# Autodesk Inventor assembly: Arm 2.0 Assembly
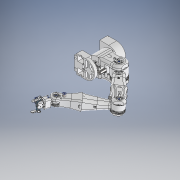
[picture p0: Inventor's stored thumbnail of the model, 180x180]
Saved by Autodesk Inventor 2017 SP1 (Build 210196100, 196)
## iProperties
Created: 2017-09-28
Part Number: Arm 2.0 Assembly
Document SubType Name: Assembly
Designer: Zach
Author: Zach
## Documents named in this file (62)
- C:\Users\Zach\Documents\GitHub\tr1\src\Body\Arm 2.0 Assembly\Arm 2.0 Assembly.iam
- C:\Users\Zach\Documents\GitHub\tr1\src\Body\Arm 2.0 Assembly\Steel Rod 8mm x 135mm.ipt
- C:\Users\Zach\Documents\GitHub\tr1\lib\22x8x8mm Bearing.ipt
- C:\Users\Zach\Documents\GitHub\tr1\src\Body\Arm 2.0 Assembly\AA004.ipt
- C:\Users\Zach\Documents\GitHub\tr1\lib\QS12MM250\QS12MM250.ipt
- C:\Users\Zach\Documents\GitHub\tr1\src\Body\Arm 2.0 Assembly\Steel Rod 8mm x 100mm.ipt
- C:\Users\Zach\Documents\GitHub\tr1\src\Body\Arm 2.0 Assembly\AA013.ipt
- C:\Users\Zach\Documents\GitHub\tr1\src\Body\Arm 2.0 Assembly\AA014.ipt
- C:\Users\Zach\Documents\GitHub\tr1\lib\12V DC Motor 378-1.ipt
- C:\Users\Zach\Documents\Inventor\Content Center Files\R2017\en-US\ISO 4017(1)\ISO 4017 - M5 x 20 - ISO.ipt
- C:\Users\Zach\Documents\GitHub\tr1\src\Body\Arm 2.0 Assembly\Steel Rod 8mm x 80mm.ipt
- C:\Users\Zach\Documents\GitHub\BCN3D-Moveo\Autodesk Inventor files\Gripper B Assembly.iam
- C:\Users\Zach\Documents\Inventor\Content Center Files\R2017\en-US\CNS 4320\CNS 4320 - M8 x 1 x 100.ipt
- C:\Users\Zach\Documents\GitHub\tr1\lib\AS 1110 - M8 x 150.ipt
- C:\Users\Zach\Documents\GitHub\tr1\lib\8mm Hub.ipt
- C:\Users\Zach\Documents\GitHub\tr1\src\Body\Arm 2.0 Assembly\Arm 2.0 Assembly\Design Accelerator\Spur Gears5.iam
- C:\Users\Zach\Documents\GitHub\tr1\lib\4mm mounting hub.ipt
- C:\Users\Zach\Documents\GitHub\tr1\lib\6201RS\6201RS.ipt
- C:\Users\Zach\Documents\GitHub\tr1\lib\U51105\U51105.ipt
- C:\Users\Zach\Documents\GitHub\tr1\src\Body\Arm 2.0 Assembly\AA031.ipt
- C:\Users\Zach\Documents\GitHub\tr1\src\Body\Arm 2.0 Assembly\AA034.ipt
- C:\Users\Zach\Documents\GitHub\tr1\src\Body\Arm 2.0 Assembly\Arm 2.0 Assembly\Design Accelerator\Spur Gears6.iam
- C:\Users\Zach\Documents\GitHub\tr1\src\Body\Arm 2.0 Assembly\AA008c.ipt
- C:\Users\Zach\Documents\GitHub\tr1\src\Body\Arm 2.0 Assembly\AA008d.ipt
- C:\Users\Zach\Documents\GitHub\tr1\src\Body\Arm 2.0 Assembly\AA035.ipt
- C:\Users\Zach\Documents\GitHub\tr1\src\Body\Arm 2.0 Assembly\Arm 2.0 Assembly\Design Accelerator\Spur Gears7.iam
- C:\Users\Zach\Documents\GitHub\tr1\src\Body\Arm 2.0 Assembly\AA036.ipt
- C:\Users\Zach\Documents\GitHub\tr1\src\Body\Arm 2.0 Assembly\AA037.ipt
- C:\Users\Zach\Documents\GitHub\tr1\src\Body\Arm 2.0 Assembly\AA016b.ipt
- C:\Users\Zach\Documents\GitHub\tr1\src\Body\Arm 2.0 Assembly\AA005b.ipt
- C:\Users\Zach\Documents\GitHub\tr1\src\Body\Arm 2.0 Assembly\AA006b.ipt
- C:\Users\Zach\Documents\GitHub\tr1\src\Body\Arm 2.0 Assembly\AA001c.ipt
- C:\Users\Zach\Documents\GitHub\tr1\lib\uxcell 12V 5RPM 8mm Worm Gear Motor\uxcell 12V 5RPM 8mm Worm Gear Motor.ipt
- C:\Users\Zach\Documents\GitHub\tr1\lib\Bourns ACE 128\Bourns ACE 128.ipt
- C:\Users\Zach\Documents\GitHub\tr1\src\Body\Arm 2.0 Assembly\Arm 2.0 Assembly\Design Accelerator\Spur Gears8.iam
- C:\Users\Zach\Documents\GitHub\tr1\src\Body\Arm 2.0 Assembly\Arm 2.0 Assembly\Design Accelerator\Spur Gears11.iam
- C:\Users\Zach\Documents\GitHub\tr1\src\Body\Arm 2.0 Assembly\Arm 2.0 Assembly\Design Accelerator\Spur Gears9.iam
- C:\Users\Zach\Documents\GitHub\tr1\src\Body\Arm 2.0 Assembly\AA010b.ipt
- C:\Users\Zach\Documents\GitHub\tr1\lib\uxcell 12V 6RPM 6mm Worm Gear Motor\uxcell 12V 6RPM 6mm Worm Gear Motor.ipt
- C:\Users\Zach\Documents\GitHub\tr1\src\Body\Arm 2.0 Assembly\Arm 2.0 Assembly\Design Accelerator\Spur Gears10.iam
- C:\Users\Zach\Documents\GitHub\tr1\src\Body\Arm 2.0 Assembly\Arm 2.0 Assembly\Design Accelerator\Spur Gears12.iam
- C:\Users\Zach\Documents\GitHub\tr1\src\Body\Arm 2.0 Assembly\AA041.ipt
- C:\Users\Zach\Documents\GitHub\tr1\src\Body\Arm 2.0 Assembly\AA042.ipt
- C:\Users\Zach\Documents\Inventor\Content Center Files\R2017\en-US\ISO 7045  H\ISO 7045 - M3 x 8 - 4.8 - H - ISO.ipt
- C:\Users\Zach\Documents\GitHub\tr1\src\Body\Arm 2.0 Assembly\AA043.ipt
- C:\Users\Zach\Documents\GitHub\tr1\src\Body\Arm 2.0 Assembly\AA044.ipt
- C:\Users\Zach\Documents\GitHub\tr1\src\Body\Arm 2.0 Assembly\AA045.ipt
- C:\Users\Zach\Documents\GitHub\tr1\src\Body\Arm 2.0 Assembly\Arm 2.0 Assembly\Design Accelerator\Spur Gears13.iam
- C:\Users\Zach\Documents\GitHub\tr1\src\Body\Arm 2.0 Assembly\Arm 2.0 Assembly\Design Accelerator\Spur Gears16.iam
- C:\Users\Zach\Documents\GitHub\tr1\src\Body\Arm 2.0 Assembly\AA046.ipt
- C:\Users\Zach\Documents\GitHub\tr1\lib\MG995.ipt
- C:\Users\Zach\Documents\GitHub\tr1\lib\Servo Mounting Hub.ipt
- C:\Users\Zach\Documents\GitHub\tr1\src\Body\Arm 2.0 Assembly\AA047.ipt
- C:\Users\Zach\Documents\GitHub\tr1\src\Body\Arm 2.0 Assembly\AA048.ipt
- C:\Users\Zach\Documents\Inventor\Content Center Files\R2017\en-US\ISO 4018\ISO 4018 - M5 x 10.ipt
- C:\Users\Zach\Documents\Inventor\Content Center Files\R2017\en-US\ISO 4018\ISO 4018 - M5 x 25.ipt
- C:\Users\Zach\Documents\Inventor\Content Center Files\R2017\en-US\ISO 7045  H\ISO 7045 - M3 x 12 - 4.8 - H - ISO.ipt
- C:\Users\Zach\Documents\GitHub\tr1\src\Body\Arm 2.0 Assembly\AA049.ipt
- C:\Users\Zach\Documents\Inventor\Content Center Files\R2017\en-US\ISO 4018\ISO 4018 - M5 x 40.ipt
- C:\Users\Zach\Documents\Inventor\Content Center Files\R2017\en-US\ISO 4035(2)\ISO 4035 - M5 - ISO.ipt
- C:\Users\Zach\Documents\Inventor\Content Center Files\R2017\en-US\ISO 4018\ISO 4018 - M5 x 35.ipt
- C:\Users\Zach\Documents\Inventor\Content Center Files\R2017\en-US\ISO 4762(2)\ISO 4762 - M4 x 10ISO.ipt
## Components (204 placed, 61 different names)
1. AA001c:1 — Mate:554, Mate:555, Mate:556, Mate:557, Mate:560, Flush:18, Mate:562, Mate:563, Mate:564, Mate:565, Mate:566, Mate:567, Mate:568, Mate:569, Mate:570, Mate:571, Mate:572, Mate:573, Mate:574, Mate:576, Mate:578, Mate:581, Angle:1, Mate:592, Mate:602, Mate:834, Mate:835, Mate:836, Mate:837, Mate:895, Mate:905, Mate:906
2. AA004:1 — Mate:23, Mate:345, Mate:347, Mate:350, Mate:357, Mate:554, Mate:555, Mate:556, Mate:590, Mate:591, Mate:826
3. AA005b:1 — Mate:537, Mate:538, Mate:539, Mate:541, Mate:542, Mate:543, Mate:806, Mate:807, Mate:808, Mate:809, Mate:838, Mate:909, Mate:910
4. AA006b:1 — Mate:544, Mate:583, Mate:584, Angle:2, Mate:588, Mate:593, Mate:594, Mate:598, Mate:599, Mate:600, Mate:609, Mate:802, Mate:803, Mate:804, Mate:805, Mate:838
5. AA008c:1 — Mate:449, Mate:450, Mate:451, Mate:452, Mate:453, Mate:454, Mate:463, Mate:464, Mate:466, Mate:467, Mate:481, Mate:616, Mate:662, Mate:663, Mate:751
6. AA008d:1 — Mate:455, Mate:456, Mate:457, Mate:461, Mate:463, Mate:464, Mate:466, Mate:467, Mate:614, Angle:4, Mate:635, Mate:662, Mate:663, Mate:697, Mate:699, Mate:751, Mate:846, Mate:847, Mate:848, Mate:849, Mate:854, Mate:855, Mate:856, Mate:857, Flush:22, Flush:23, Mate:858, Mate:859, Mate:925, Mate:926
7. AA010b:1 — Mate:615, Mate:616, Mate:617, Mate:618, Mate:620, Mate:621, Mate:623, Mate:624, Mate:625, Mate:626, Mate:628, Mate:630, Mate:632, Mate:633, Mate:634, Mate:636, Mate:637, Angle:6, Mate:642, Flush:20, Mate:648, Mate:650, Mate:927, Mate:928, Mate:929, Mate:930, Mate:931, Mate:932, Mate:948, Mate:949
8. AA013:2 — Mate:142, Mate:143, Mate:144, Mate:145, Mate:146, Mate:147, Mate:563, Mate:564, Mate:565
9. AA014:2 — Mate:628, Mate:629, Mate:630, Mate:976, Mate:977, Mate:978, Mate:979, Mate:980, Mate:981
10. AA016b:1 — Mate:518, Mate:519, Mate:520, Mate:521, Mate:525, Mate:526, Mate:527, Mate:529, Mate:530, Mate:664, Mate:665, Mate:667, Mate:668, Mate:669, Angle:7, Mate:671, Mate:673, Mate:675, Mate:676, Mate:677, Mate:877, Mate:878
11. AA031:1 — Mate:366, Mate:367, Mate:523, Mate:524, Mate:954, Mate:955, Mate:956, Mate:957
12. AA034:1 — Mate:529, Mate:534, Mate:535, Mate:700, Mate:701, Mate:709, Mate:879, Mate:880, Mate:881, Mate:882, Mate:883, Mate:884, Mate:885, Mate:886, Mate:964, Mate:965, Mate:966, Mate:967, Mate:968, Mate:969, Mate:970, Mate:971, Mate:972, Mate:973, Mate:974, Mate:975
13. AA035:1 — Mate:477, Mate:479, Mate:481, Mate:557, Mate:601, Mate:652, Mate:653, Mate:697, Mate:699, Mate:851, Mate:853
14. AA036:1 — Mate:498, Mate:501, Mate:502, Mate:511, Mate:698, Mate:868, Mate:871, Mate:872, Mate:939
15. AA037:1 — Mate:501, Mate:502, Mate:514, Mate:515, Mate:516, Mate:517, Mate:518, Mate:519, Mate:520, Mate:530, Mate:664, Mate:665, Mate:698, Mate:866, Mate:867, Mate:873, Mate:874, Mate:875, Mate:876, Flush:25, Flush:26, Mate:950, Mate:951, Mate:952, Mate:953
16. AA041:1 — Mate:675, Mate:676, Mate:677, Mate:682, Mate:683, Mate:684, Mate:685
17. AA042:1 — Mate:678, Mate:679, Mate:686, Mate:687, Angle:14
18. AA043:1 — Mate:688, Mate:689, Angle:8
19. AA043:2 — Mate:693, Mate:694, Angle:10
20. AA043:3 — Mate:742, Mate:743, Angle:13
21. AA044:1 — Mate:691, Mate:692, Angle:9
22. AA044:2 — Mate:695, Mate:696, Angle:11, Mate:892, Mate:893
23. AA045:2 — Mate:700, Mate:701, Mate:702, Mate:703, Mate:704, Mate:705, Mate:706, Mate:708, Flush:21, Mate:709, Mate:711, Mate:713, Mate:715, Mate:717, Mate:718, Angle:12, Mate:719, Mate:720, Mate:723, Mate:725, Mate:780, Mate:781, Mate:784, Mate:785
24. AA046:1 — Mate:727, Mate:728, Mate:731, Mate:735, Mate:736, Mate:737, Mate:752, Mate:756, Mate:757, Mate:758, Mate:759, Mate:760, Mate:761, Mate:762, Mate:763
25. AA047:1 — Mate:735, Mate:736, Mate:737, Mate:738, Mate:739, Mate:740, Mate:753, Mate:754, Mate:755, Mate:800, Mate:801
26. AA048:1 — Mate:744, Mate:745, Mate:746, Mate:747, Mate:748, Mate:749
27. AA049:1 — Mate:783, Mate:784, Mate:785, Mate:786, Mate:787, Mate:788, Mate:789, Mate:790, Mate:791
28. Gripper B Assembly:1 [sub-assembly] — Mate:747, Mate:748, Mate:749
29. 22x8x8mm Bearing:1 — Mate:433, Mate:560
30. 22x8x8mm Bearing:2 — Mate:437, Mate:562
31. 22x8x8mm Bearing:3 — Mate:57, Mate:620, Mate:626, Mate:645
32. 22x8x8mm Bearing:4 — Mate:621, Mate:629, Mate:642
33. 22x8x8mm Bearing:5 — Mate:186, Mate:708
34. 22x8x8mm Bearing:6 — Mate:187, Mate:719
35. 22x8x8mm Bearing:7 — Mate:264, Mate:526
36. 22x8x8mm Bearing:8 — Mate:527, Mate:528
37. 22x8x8mm Bearing:13 — Mate:451, Mate:452
38. 22x8x8mm Bearing:14 — Mate:449, Mate:450
39. QS12MM250:1 — Mate:23, Mate:344, Mate:346, Mate:348, Mate:354, Mate:537, Mate:544, Mate:585, Mate:593, Mate:594, Mate:597
40. Steel Rod 8mm x 135mm:1 — Mate:433, Mate:437, Mate:476, Mate:477, Flush:18, Mate:575, Mate:651
41. Steel Rod 8mm x 100mm:1 — Mate:57, Mate:491, Mate:498, Flush:20, Mate:644, Mate:649
42. Steel Rod 8mm x 80mm:1 — Mate:186, Mate:187, Mate:706, Flush:21, Mate:710, Mate:721, Mate:724, Mate:730, Mate:783
43. 12V DC Motor 378-1:3 — Mate:702, Mate:703, Mate:704, Mate:705, Mate:712, Mate:714, Mate:778, Mate:779
44. 12V DC Motor 378-1:4 — Mate:514, Mate:515, Mate:516, Mate:522
45. 12V DC Motor 378-1:6 — Mate:340, Mate:342, Mate:538, Mate:539, Mate:540, Mate:543, Mate:907, Mate:908
46. 12V DC Motor 378-1:7 — Mate:455, Mate:456, Mate:457, Mate:460, Mate:610, Mate:923, Mate:924
47. uxcell 12V 6RPM 6mm Worm Gear Motor:1 — Mate:632, Mate:633, Mate:634, Mate:946, Mate:947
48. uxcell 12V 5RPM 8mm Worm Gear Motor:1 — Mate:568, Mate:569, Mate:570, Mate:571, Mate:572, Mate:894, Mate:903, Mate:904
49. 6201RS:1 — Mate:346, Mate:347
50. 6201RS:2 — Mate:357, Mate:597
51. U51105:1 — Mate:348, Mate:349, Mate:542
52. U51105:2 — Mate:354, Mate:608, Mate:609
53. 8mm Hub:2 — Mate:368, Mate:531, Mate:534, Mate:535
54. 8mm Hub:3 — Mate:617, Mate:618, Mate:690, Mate:933, Mate:934, Mate:935, Mate:936, Mate:937, Mate:938
55. 8mm Hub:4 — Mate:580, Mate:581, Mate:582
56. 8mm Hub:5 — Mate:644, Mate:645, Mate:646
57. 8mm Hub:6 — Mate:651, Mate:652, Mate:653, Mate:911, Mate:912, Mate:913, Mate:914, Mate:915, Mate:916
58. 8mm Hub:7 — Mate:666, Mate:667, Mate:674
59. 8mm Hub:8 — Mate:720, Mate:721, Mate:726
60. 8mm Hub:9 — Mate:727, Mate:728, Mate:730, Mate:756, Mate:764, Mate:765, Mate:766, Mate:767, Mate:768, Mate:769
61. 8mm Hub:10 — Mate:894, Mate:895, Mate:896
62. 4mm mounting hub:1 — Mate:340, Mate:540, Mate:541, Mate:887
63. 4mm mounting hub:3 — Mate:366, Mate:367, Mate:517, Mate:522, Mate:523, Mate:524
64. 4mm mounting hub:5 — Mate:513, Mate:622, Mate:623
65. 4mm mounting hub:7 — Mate:460, Mate:461, Mate:611, Mate:613
66. 4mm mounting hub:8 — Mate:714, Mate:715, Mate:716, Mate:782
67. Servo Mounting Hub:1 — Mate:733, Mate:734, Mate:738, Mate:739, Mate:740, Mate:792, Mate:793, Mate:794, Mate:795, Mate:796, Mate:797, Mate:798, Mate:799
68. Bourns ACE 128:1 — Mate:573, Mate:574, Mate:577, Angle:1, Mate:693, Mate:694
69. Bourns ACE 128:2 — Mate:583, Mate:584, Angle:2, Mate:587, Mate:695, Mate:696
70. Bourns ACE 128:3 — Mate:612, Mate:614, Angle:4, Mate:635, Mate:691, Mate:692
71. Bourns ACE 128:4 — Mate:636, Mate:637, Angle:6, Mate:647, Mate:688, Mate:689
72. Bourns ACE 128:5 — Mate:668, Mate:669, Angle:7, Mate:672, Mate:678, Mate:679
73. Bourns ACE 128:6 — Mate:717, Mate:718, Angle:12, Mate:722, Mate:742, Mate:743
74. AASG01 [sub-assembly] — Mate:342, Mate:344, Mate:345, Mate:349, Mate:350, Mate:810, Mate:811, Mate:812, Mate:813, Mate:814, Mate:815, Mate:816, Mate:817, Mate:818, Mate:819, Mate:820, Mate:821, Mate:887, Mate:888, Mate:889, Mate:890, Mate:891
75. AASG02 [sub-assembly] — Mate:476, Mate:479, Mate:566, Mate:567, Mate:601, Mate:602, Mate:839, Mate:841, Mate:842, Mate:843, Mate:844, Mate:845, Mate:896, Mate:897, Mate:898, Mate:899, Mate:900, Mate:901, Mate:902
76. AASG03 [sub-assembly] — Mate:491, Mate:511, Mate:513, Mate:622, Mate:624, Mate:625, Mate:860, Mate:861, Mate:862, Mate:863, Mate:864, Mate:865, Mate:940, Mate:941, Mate:942, Mate:943, Mate:944, Mate:945
77. AASG04 [sub-assembly] — Mate:575, Mate:576, Mate:577, Mate:578, Mate:580, Mate:582, Angle:10, Mate:917, Mate:918, Mate:919, Mate:920, Mate:921, Mate:922
78. AASG05 [sub-assembly] — Mate:585, Mate:587, Mate:588, Mate:590, Mate:591, Mate:592, Mate:608, Angle:11, Mate:822, Mate:823, Mate:824, Mate:825, Mate:827, Mate:828, Mate:829, Mate:830, Mate:831, Mate:832, Mate:833
79. AASG06 [sub-assembly] — Mate:610, Mate:611, Mate:612, Mate:613, Angle:5, Angle:9
80. AASG07 [sub-assembly] — Mate:646, Mate:647, Mate:648, Mate:649, Mate:650, Angle:8, Mate:958, Mate:959, Mate:960, Mate:961, Mate:962, Mate:963
81. AASG08 [sub-assembly] — Mate:670, Mate:671, Mate:672, Mate:673, Mate:674, Mate:680, Mate:681, Angle:14
82. AASG09 [sub-assembly] — Mate:710, Mate:711, Mate:712, Mate:713, Mate:716, Mate:731, Mate:757, Mate:770, Mate:771, Mate:772, Mate:773, Mate:774, Mate:775, Mate:776, Mate:777, Mate:782
83. AASG10 [sub-assembly] — Mate:722, Mate:723, Mate:724, Mate:725, Mate:726, Angle:13
84. MG995:1 — Mate:733, Mate:734, Mate:744, Mate:745, Mate:746
85. CNS 4320 M8 x 100:1 — Mate:264, Mate:368, Mate:521, Mate:525, Mate:528, Mate:531, Mate:666, Mate:670
86. AS 1110 - Metric M8 x 150:2 — Mate:453, Mate:454, Angle:5, Mate:615, Mate:690
87. ISO 7045 H M3 x 8 - 4.8 - H:1 — Mate:680, Mate:681
88. ISO 7045 H M3 x 8 - 4.8 - H:2 — Mate:682, Mate:685
89. ISO 7045 H M3 x 8 - 4.8 - H:3 — Mate:683, Mate:684
90. ISO 7045 H M3 x 8 - 4.8 - H:4 — Mate:686, Mate:687
91. ISO 7045 H M3 x 8 - 4.8 - H:5 — Mate:778, Mate:780
92. ISO 7045 H M3 x 8 - 4.8 - H:6 — Mate:779, Mate:781
93. ISO 7045 H M3 x 8 - 4.8 - H:7 — Mate:795, Mate:799
94. ISO 7045 H M3 x 8 - 4.8 - H:8 — Mate:794, Mate:798
95. ISO 7045 H M3 x 8 - 4.8 - H:9 — Mate:792, Mate:796
96. ISO 7045 H M3 x 8 - 4.8 - H:10 — Mate:793, Mate:797
97. ISO 7045 H M3 x 8 - 4.8 - H:11 — Mate:800, Mate:801
98. ISO 7045 H M3 x 8 - 4.8 - H:12 — Mate:892, Mate:893
99. ISO 7045 H M3 x 8 - 4.8 - H:13 — Mate:897, Mate:900
100. ISO 7045 H M3 x 8 - 4.8 - H:14 — Mate:898, Mate:901
101. ISO 7045 H M3 x 8 - 4.8 - H:15 — Mate:899, Mate:902
102. ISO 7045 H M3 x 8 - 4.8 - H:16 — Mate:908, Mate:910
103. ISO 7045 H M3 x 8 - 4.8 - H:17 — Mate:907, Mate:909
104. ISO 7045 H M3 x 8 - 4.8 - H:18 — Mate:923, Mate:925
105. ISO 7045 H M3 x 8 - 4.8 - H:19 — Mate:924, Mate:926
106. ISO 7045 H M3 x 8 - 4.8 - H:20 — Mate:951, Mate:953
107. ISO 7045 H M3 x 8 - 4.8 - H:21 — Mate:950, Mate:952
108. ISO 7045 H M3 x 8 - 4.8 - H:23 — Mate:955, Mate:957
109. ISO 7045 H M3 x 8 - 4.8 - H:22 — Mate:954, Mate:956
110. ISO 7045 H M3 x 8 - 4.8 - H:24 — Mate:960, Mate:963
111. ISO 7045 H M3 x 8 - 4.8 - H:25 — Mate:958, Mate:962
112. ISO 7045 H M3 x 8 - 4.8 - H:26 — Mate:959, Mate:961
113. ISO 7045 H M3 x 8 - 4.8 - H:27 — Mate:965, Mate:972
114. ISO 7045 H M3 x 8 - 4.8 - H:28 — Mate:964, Mate:973
115. ISO 7045 H M3 x 8 - 4.8 - H:29 — Mate:966, Mate:971
116. ISO 7045 H M3 x 8 - 4.8 - H:30 — Mate:967, Mate:970
117. ISO 7045 H M3 x 8 - 4.8 - H:31 — Mate:969, Mate:975
118. ISO 7045 H M3 x 8 - 4.8 - H:32 — Mate:968, Mate:974
119. ISO 7045 H M3 x 12 - 4.8 - H:1 — Mate:765, Mate:767
120. ISO 7045 H M3 x 12 - 4.8 - H:3 — Mate:764, Mate:769
121. ISO 7045 H M3 x 12 - 4.8 - H:2 — Mate:766, Mate:768
122. ISO 7045 H M3 x 12 - 4.8 - H:4 — Mate:770, Mate:775
123. ISO 7045 H M3 x 12 - 4.8 - H:5 — Mate:771, Mate:774
124. ISO 7045 H M3 x 12 - 4.8 - H:6 — Mate:773, Mate:777
125. ISO 7045 H M3 x 12 - 4.8 - H:7 — Mate:772, Mate:776
126. ISO 7045 H M3 x 12 - 4.8 - H:8 — Mate:889, Mate:890
127. ISO 7045 H M3 x 12 - 4.8 - H:9 — Mate:888, Mate:891
128. ISO 7045 H M3 x 12 - 4.8 - H:10 — Mate:911, Mate:914
129. ISO 7045 H M3 x 12 - 4.8 - H:11 — Mate:913, Mate:915
130. ISO 7045 H M3 x 12 - 4.8 - H:12 — Mate:912, Mate:916
131. ISO 7045 H M3 x 12 - 4.8 - H:13 — Mate:919, Mate:920
132. ISO 7045 H M3 x 12 - 4.8 - H:14 — Mate:917, Mate:921
133. ISO 7045 H M3 x 12 - 4.8 - H:15 — Mate:918, Mate:922
134. ISO 7045 H M3 x 12 - 4.8 - H:16 — Mate:929, Mate:936
135. ISO 7045 H M3 x 12 - 4.8 - H:17 — Mate:932, Mate:934
136. ISO 7045 H M3 x 12 - 4.8 - H:18 — Mate:931, Mate:935
137. ISO 7045 H M3 x 12 - 4.8 - H:19 — Mate:930, Mate:933
138. ISO 7045 H M3 x 12 - 4.8 - H:20 — Mate:928, Mate:937
139. ISO 7045 H M3 x 12 - 4.8 - H:21 — Mate:927, Mate:938
140. ISO 7045 H M3 x 12 - 4.8 - H:22 — Mate:942, Mate:943
141. ISO 7045 H M3 x 12 - 4.8 - H:23 — Mate:941, Mate:944
142. ISO 7045 H M3 x 12 - 4.8 - H:24 — Mate:940, Mate:945
143. ISO 4762 M4 x 10:1 — Mate:903, Mate:905
144. ISO 4762 M4 x 10:2 — Mate:904, Mate:906
145. ISO 4762 M4 x 10:3 — Mate:946, Mate:949
146. ISO 4762 M4 x 10:4 — Mate:947, Mate:948
147. ISO 4035 M5:1 — Mate:850, Mate:851
148. ISO 4035 M5:2 — Mate:852, Mate:853
149. ISO 4035 M5:3 — Mate:869, Mate:872
150. ISO 4035 M5:4 — Mate:870, Mate:871
151. ISO 4018 M5 x 10:1 — Mate:754, Mate:755
152. ISO 4018 M5 x 10:2 — Mate:752, Mate:753
153. ISO 4018 M5 x 10:3 — Mate:787, Mate:790
154. ISO 4018 M5 x 10:4 — Mate:788, Mate:791
155. ISO 4018 M5 x 10:5 — Mate:786, Mate:789
156. ISO 4017 M5 x 20:1 — Mate:146, Mate:147
157. ISO 4017 M5 x 20:2 — Mate:144, Mate:145
158. ISO 4017 M5 x 20:3 — Mate:142, Mate:143
159. ISO 4017 M5 x 20:4 — Mate:978, Mate:980
160. ISO 4017 M5 x 20:5 — Mate:977, Mate:979
161. ISO 4017 M5 x 20:6 — Mate:976, Mate:981
162. ISO 4018 M5 x 25:1 — Mate:758, Mate:761
163. ISO 4018 M5 x 25:2 — Mate:759, Mate:763
164. ISO 4018 M5 x 25:3 — Mate:760, Mate:762
165. ISO 4018 M5 x 25:7 — Mate:802, Mate:803
166. ISO 4018 M5 x 25:8 — Mate:804, Mate:805
167. ISO 4018 M5 x 25:9 — Mate:806, Mate:808
168. ISO 4018 M5 x 25:10 — Mate:807, Mate:809
169. ISO 4018 M5 x 25:11 — Mate:812, Mate:820
170. ISO 4018 M5 x 25:12 — Mate:810, Mate:816
171. ISO 4018 M5 x 25:13 — Mate:811, Mate:821
172. ISO 4018 M5 x 25:14 — Mate:814, Mate:817
173. ISO 4018 M5 x 25:15 — Mate:813, Mate:819
174. ISO 4018 M5 x 25:16 — Mate:815, Mate:818
175. ISO 4018 M5 x 25:17 — Mate:823, Mate:831
176. ISO 4018 M5 x 25:18 — Mate:824, Mate:829
177. ISO 4018 M5 x 25:19 — Mate:825, Mate:832
178. ISO 4018 M5 x 25:20 — Mate:827, Mate:828
179. ISO 4018 M5 x 25:21 — Mate:826, Mate:833
180. ISO 4018 M5 x 25:22 — Mate:822, Mate:830
181. ISO 4018 M5 x 25:23 — Mate:836, Mate:837
182. ISO 4018 M5 x 25:24 — Mate:834, Mate:835
183. ISO 4018 M5 x 25:25 — Mate:839, Mate:845
184. ISO 4018 M5 x 25:27 — Mate:841, Mate:844
185. ISO 4018 M5 x 25:28 — Mate:842, Mate:843
186. ISO 4018 M5 x 25:29 — Mate:854, Mate:858
187. ISO 4018 M5 x 25:30 — Mate:856, Flush:23
188. ISO 4018 M5 x 25:31 — Mate:857, Flush:22
189. ISO 4018 M5 x 25:32 — Mate:855, Mate:859
190. ISO 4018 M5 x 25:33 — Mate:860, Mate:865, Mate:939
191. ISO 4018 M5 x 25:34 — Mate:862, Mate:863
192. ISO 4018 M5 x 25:35 — Mate:861, Mate:864
193. ISO 4018 M5 x 25:36 — Mate:876, Mate:878
194. ISO 4018 M5 x 25:37 — Mate:875, Mate:877
195. ISO 4018 M5 x 25:38 — Mate:874, Flush:26
196. ISO 4018 M5 x 25:39 — Mate:873, Flush:25
197. ISO 4018 M5 x 25:40 — Mate:882, Mate:883
198. ISO 4018 M5 x 25:41 — Mate:880, Mate:886
199. ISO 4018 M5 x 25:42 — Mate:879, Mate:885
200. ISO 4018 M5 x 25:43 — Mate:881, Mate:884
201. ISO 4018 M5 x 35:1 — Mate:866, Mate:867, Flush:24, Mate:869
202. ISO 4018 M5 x 35:2 — Mate:868, Flush:24, Mate:870
203. ISO 4018 M5 x 40:1 — Mate:846, Mate:848, Mate:850
204. ISO 4018 M5 x 40:2 — Mate:847, Mate:849, Mate:852
## Relationships (494: Mate 473, Angle 13, Flush 8)
- Mate:23: AA004:1 ↔ QS12MM250:1
- Mate:57: 22x8x8mm Bearing:3 ↔ Steel Rod 8mm x 100mm:1
- Mate:142: AA013:2 ↔ ISO 4017 M5 x 20:3
- Mate:143: AA013:2 ↔ ISO 4017 M5 x 20:3
- Mate:144: AA013:2 ↔ ISO 4017 M5 x 20:2
- Mate:145: AA013:2 ↔ ISO 4017 M5 x 20:2
- Mate:146: AA013:2 ↔ ISO 4017 M5 x 20:1
- Mate:147: AA013:2 ↔ ISO 4017 M5 x 20:1
- Mate:186: 22x8x8mm Bearing:5 ↔ Steel Rod 8mm x 80mm:1
- Mate:187: 22x8x8mm Bearing:6 ↔ Steel Rod 8mm x 80mm:1
- Mate:264: 22x8x8mm Bearing:7 ↔ CNS 4320 M8 x 100:1
- Mate:340: 12V DC Motor 378-1:6 ↔ 4mm mounting hub:1
- Mate:342: 12V DC Motor 378-1:6 ↔ AASG01
- Mate:344: QS12MM250:1 ↔ AASG01
- Mate:345: AA004:1 ↔ AASG01
- Mate:346: QS12MM250:1 ↔ 6201RS:1
- Mate:347: AA004:1 ↔ 6201RS:1
- Mate:348: QS12MM250:1 ↔ U51105:1
- Mate:349: U51105:1 ↔ AASG01
- Mate:350: AA004:1 ↔ AASG01
- Mate:354: QS12MM250:1 ↔ U51105:2
- Mate:357: AA004:1 ↔ 6201RS:2
- Mate:366: AA031:1 ↔ 4mm mounting hub:3
- Mate:367: AA031:1 ↔ 4mm mounting hub:3
- Mate:368: 8mm Hub:2 ↔ CNS 4320 M8 x 100:1
- Mate:433: 22x8x8mm Bearing:1 ↔ Steel Rod 8mm x 135mm:1
- Mate:437: 22x8x8mm Bearing:2 ↔ Steel Rod 8mm x 135mm:1
- Mate:449: AA008c:1 ↔ 22x8x8mm Bearing:14
- Mate:450: AA008c:1 ↔ 22x8x8mm Bearing:14
- Mate:451: AA008c:1 ↔ 22x8x8mm Bearing:13
- Mate:452: AA008c:1 ↔ 22x8x8mm Bearing:13
- Mate:453: AA008c:1 ↔ AS 1110 - Metric M8 x 150:2
- Mate:454: AA008c:1 ↔ AS 1110 - Metric M8 x 150:2
- Mate:455: AA008d:1 ↔ 12V DC Motor 378-1:7
- Mate:456: AA008d:1 ↔ 12V DC Motor 378-1:7
- Mate:457: AA008d:1 ↔ 12V DC Motor 378-1:7
- Mate:460: 12V DC Motor 378-1:7 ↔ 4mm mounting hub:7
- Mate:461: AA008d:1 ↔ 4mm mounting hub:7
- Mate:463: AA008c:1 ↔ AA008d:1
- Mate:464: AA008c:1 ↔ AA008d:1
- Mate:466: AA008c:1 ↔ AA008d:1
- Mate:467: AA008c:1 ↔ AA008d:1
- Mate:476: Steel Rod 8mm x 135mm:1 ↔ AASG02
- Mate:477: AA035:1 ↔ Steel Rod 8mm x 135mm:1
- Mate:479: AA035:1 ↔ AASG02
- Mate:481: AA008c:1 ↔ AA035:1
- Mate:491: Steel Rod 8mm x 100mm:1 ↔ AASG03
- Mate:498: AA036:1 ↔ Steel Rod 8mm x 100mm:1
- Mate:501: AA036:1 ↔ AA037:1
- Mate:502: AA036:1 ↔ AA037:1
- Mate:511: AA036:1 ↔ AASG03
- Mate:513: 4mm mounting hub:5 ↔ AASG03
- Mate:514: AA037:1 ↔ 12V DC Motor 378-1:4
- Mate:515: AA037:1 ↔ 12V DC Motor 378-1:4
- Mate:516: AA037:1 ↔ 12V DC Motor 378-1:4
- Mate:517: AA037:1 ↔ 4mm mounting hub:3
- Mate:518: AA016b:1 ↔ AA037:1
- Mate:519: AA016b:1 ↔ AA037:1
- Mate:520: AA016b:1 ↔ AA037:1
- Mate:521: AA016b:1 ↔ CNS 4320 M8 x 100:1
- Mate:522: 12V DC Motor 378-1:4 ↔ 4mm mounting hub:3
- Mate:523: AA031:1 ↔ 4mm mounting hub:3
- Mate:524: AA031:1 ↔ 4mm mounting hub:3
- Mate:525: AA016b:1 ↔ CNS 4320 M8 x 100:1
- Mate:526 (0.5 mm): AA016b:1 ↔ 22x8x8mm Bearing:7
- Mate:527 (0.5 mm): AA016b:1 ↔ 22x8x8mm Bearing:8
- Mate:528: 22x8x8mm Bearing:8 ↔ CNS 4320 M8 x 100:1
- Mate:529: AA016b:1 ↔ AA034:1
- Mate:530: AA016b:1 ↔ AA037:1
- Mate:531: 8mm Hub:2 ↔ CNS 4320 M8 x 100:1
- Mate:534: AA034:1 ↔ 8mm Hub:2
- Mate:535: AA034:1 ↔ 8mm Hub:2
- Mate:537: AA005b:1 ↔ QS12MM250:1
- Mate:538: AA005b:1 ↔ 12V DC Motor 378-1:6
- Mate:539: AA005b:1 ↔ 12V DC Motor 378-1:6
- Mate:540: 12V DC Motor 378-1:6 ↔ 4mm mounting hub:1
- Mate:541: AA005b:1 ↔ 4mm mounting hub:1
- Mate:542: AA005b:1 ↔ U51105:1
- Mate:543: AA005b:1 ↔ 12V DC Motor 378-1:6
- Mate:544: AA006b:1 ↔ QS12MM250:1
- Mate:554: AA001c:1 ↔ AA004:1
- Mate:555: AA001c:1 ↔ AA004:1
- Mate:556: AA001c:1 ↔ AA004:1
- Mate:557: AA001c:1 ↔ AA035:1
- Mate:560: AA001c:1 ↔ 22x8x8mm Bearing:1
- Flush:18: AA001c:1 ↔ Steel Rod 8mm x 135mm:1
- Mate:562: AA001c:1 ↔ 22x8x8mm Bearing:2
- Mate:563: AA001c:1 ↔ AA013:2
- Mate:564: AA001c:1 ↔ AA013:2
- Mate:565: AA001c:1 ↔ AA013:2
- Mate:566: AA001c:1 ↔ AASG02
- Mate:567 (1 mm): AA001c:1 ↔ AASG02
- Mate:568: AA001c:1 ↔ uxcell 12V 5RPM 8mm Worm Gear Motor:1
- Mate:569: AA001c:1 ↔ uxcell 12V 5RPM 8mm Worm Gear Motor:1
- Mate:570: AA001c:1 ↔ uxcell 12V 5RPM 8mm Worm Gear Motor:1
- Mate:571: AA001c:1 ↔ uxcell 12V 5RPM 8mm Worm Gear Motor:1
- Mate:572: AA001c:1 ↔ uxcell 12V 5RPM 8mm Worm Gear Motor:1
- Mate:573: AA001c:1 ↔ Bourns ACE 128:1
- Mate:574: AA001c:1 ↔ Bourns ACE 128:1
- Mate:575: Steel Rod 8mm x 135mm:1 ↔ AASG04
- Mate:576: AA001c:1 ↔ AASG04
- Mate:577: Bourns ACE 128:1 ↔ AASG04
- Mate:578: AA001c:1 ↔ AASG04
- Mate:580: 8mm Hub:4 ↔ AASG04
- Mate:581: AA001c:1 ↔ 8mm Hub:4
- Mate:582: 8mm Hub:4 ↔ AASG04
- Angle:1 (0 deg): AA001c:1 ↔ Bourns ACE 128:1
- Mate:583: AA006b:1 ↔ Bourns ACE 128:2
- Mate:584: AA006b:1 ↔ Bourns ACE 128:2
- Angle:2 (0 deg): AA006b:1 ↔ Bourns ACE 128:2
- Mate:585: QS12MM250:1 ↔ AASG05
- Mate:587: Bourns ACE 128:2 ↔ AASG05
- Mate:588: AA006b:1 ↔ AASG05
- Mate:590: AA004:1 ↔ AASG05
- Mate:591: AA004:1 ↔ AASG05
- Mate:592: AA001c:1 ↔ AASG05
- Mate:593: AA006b:1 ↔ QS12MM250:1
- Mate:594: AA006b:1 ↔ QS12MM250:1
- Mate:597: QS12MM250:1 ↔ 6201RS:2
- Mate:598: AA006b:1
- Mate:599: AA006b:1
- Mate:600: AA006b:1
- Mate:601: AA035:1 ↔ AASG02
- Mate:602 (2.5 mm): AA001c:1 ↔ AASG02
- Mate:608: U51105:2 ↔ AASG05
- Mate:609: AA006b:1 ↔ U51105:2
- Mate:610: 12V DC Motor 378-1:7 ↔ AASG06
- Mate:611: 4mm mounting hub:7 ↔ AASG06
- Mate:612: Bourns ACE 128:3 ↔ AASG06
- Mate:613: 4mm mounting hub:7 ↔ AASG06
- Mate:614: AA008d:1 ↔ Bourns ACE 128:3
- Angle:4 (0 deg): AA008d:1 ↔ Bourns ACE 128:3
- Angle:5 (0 deg): AASG06 ↔ AS 1110 - Metric M8 x 150:2
- Mate:615: AA010b:1 ↔ AS 1110 - Metric M8 x 150:2
- Mate:616: AA008c:1 ↔ AA010b:1
- Mate:617: AA010b:1 ↔ 8mm Hub:3
- Mate:618: AA010b:1 ↔ 8mm Hub:3
- Mate:620: AA010b:1 ↔ 22x8x8mm Bearing:3
- Mate:621: AA010b:1 ↔ 22x8x8mm Bearing:4
- Mate:622: 4mm mounting hub:5 ↔ AASG03
- Mate:623: AA010b:1 ↔ 4mm mounting hub:5
- Mate:624: AA010b:1 ↔ AASG03
- Mate:625: AA010b:1 ↔ AASG03
- Flush:20 (0.5 mm): AA010b:1 ↔ Steel Rod 8mm x 100mm:1
- Mate:626: AA010b:1 ↔ 22x8x8mm Bearing:3
- Mate:628: AA010b:1 ↔ AA014:2
- Mate:629: AA014:2 ↔ 22x8x8mm Bearing:4
- Mate:630: AA010b:1 ↔ AA014:2
- Mate:632: AA010b:1 ↔ uxcell 12V 6RPM 6mm Worm Gear Motor:1
- Mate:633: AA010b:1 ↔ uxcell 12V 6RPM 6mm Worm Gear Motor:1
- Mate:634: AA010b:1 ↔ uxcell 12V 6RPM 6mm Worm Gear Motor:1
- Mate:635: AA008d:1 ↔ Bourns ACE 128:3
- Mate:636: AA010b:1 ↔ Bourns ACE 128:4
- Mate:637: AA010b:1 ↔ Bourns ACE 128:4
- Angle:6 (0 deg): AA010b:1 ↔ Bourns ACE 128:4
- Mate:642: AA010b:1 ↔ 22x8x8mm Bearing:4
- Mate:644: Steel Rod 8mm x 100mm:1 ↔ 8mm Hub:5
- Mate:645: 22x8x8mm Bearing:3 ↔ 8mm Hub:5
- Mate:646: 8mm Hub:5 ↔ AASG07
- Mate:647: Bourns ACE 128:4 ↔ AASG07
- Mate:648: AA010b:1 ↔ AASG07
- Mate:649: Steel Rod 8mm x 100mm:1 ↔ AASG07
- Mate:650: AA010b:1 ↔ AASG07
- Mate:651: Steel Rod 8mm x 135mm:1 ↔ 8mm Hub:6
- Mate:652: AA035:1 ↔ 8mm Hub:6
- Mate:653: AA035:1 ↔ 8mm Hub:6
- Mate:662: AA008c:1 ↔ AA008d:1
- Mate:663: AA008c:1 ↔ AA008d:1
- Mate:664: AA016b:1 ↔ AA037:1
- Mate:665: AA016b:1 ↔ AA037:1
- Mate:666: 8mm Hub:7 ↔ CNS 4320 M8 x 100:1
- Mate:667: AA016b:1 ↔ 8mm Hub:7
- Mate:668: AA016b:1 ↔ Bourns ACE 128:5
- Mate:669: AA016b:1 ↔ Bourns ACE 128:5
- Angle:7 (0 deg): AA016b:1 ↔ Bourns ACE 128:5
- Mate:670: AASG08 ↔ CNS 4320 M8 x 100:1
- Mate:671: AA016b:1 ↔ AASG08
- Mate:672: Bourns ACE 128:5 ↔ AASG08
- Mate:673: AA016b:1 ↔ AASG08
- Mate:674: 8mm Hub:7 ↔ AASG08
- Mate:675: AA016b:1 ↔ AA041:1
- Mate:676: AA016b:1 ↔ AA041:1
- Mate:677: AA016b:1 ↔ AA041:1
- Mate:678: AA042:1 ↔ Bourns ACE 128:5
- Mate:679: AA042:1 ↔ Bourns ACE 128:5
- Mate:680: AASG08 ↔ ISO 7045 H M3 x 8 - 4.8 - H:1
- Mate:681: AASG08 ↔ ISO 7045 H M3 x 8 - 4.8 - H:1
- Mate:682: AA041:1 ↔ ISO 7045 H M3 x 8 - 4.8 - H:2
- Mate:683: AA041:1 ↔ ISO 7045 H M3 x 8 - 4.8 - H:3
- Mate:684: AA041:1 ↔ ISO 7045 H M3 x 8 - 4.8 - H:3
- Mate:685: AA041:1 ↔ ISO 7045 H M3 x 8 - 4.8 - H:2
- Mate:686: AA042:1 ↔ ISO 7045 H M3 x 8 - 4.8 - H:4
- Mate:687: AA042:1 ↔ ISO 7045 H M3 x 8 - 4.8 - H:4
- Mate:688: AA043:1 ↔ Bourns ACE 128:4
- Mate:689: AA043:1 ↔ Bourns ACE 128:4
- Angle:8 (0 deg): AA043:1 ↔ AASG07
- Mate:690: 8mm Hub:3 ↔ AS 1110 - Metric M8 x 150:2
- Mate:691: AA044:1 ↔ Bourns ACE 128:3
- Mate:692: AA044:1 ↔ Bourns ACE 128:3
- Angle:9 (0 deg): AA044:1 ↔ AASG06
- Mate:693: AA043:2 ↔ Bourns ACE 128:1
- Mate:694: AA043:2 ↔ Bourns ACE 128:1
- Angle:10 (0 deg): AA043:2 ↔ AASG04
- Mate:695: AA044:2 ↔ Bourns ACE 128:2
- Mate:696: AA044:2 ↔ Bourns ACE 128:2
- Angle:11 (0 deg): AA044:2 ↔ AASG05
- Mate:697: AA008d:1 ↔ AA035:1
- Mate:698: AA036:1 ↔ AA037:1
- Mate:699: AA008d:1 ↔ AA035:1
- Mate:700: AA034:1 ↔ AA045:2
- Mate:701: AA034:1 ↔ AA045:2
- Mate:702: AA045:2 ↔ 12V DC Motor 378-1:3
- Mate:703: AA045:2 ↔ 12V DC Motor 378-1:3
- Mate:704: AA045:2 ↔ 12V DC Motor 378-1:3
- Mate:705: AA045:2 ↔ 12V DC Motor 378-1:3
- Mate:706: AA045:2 ↔ Steel Rod 8mm x 80mm:1
- Mate:708: AA045:2 ↔ 22x8x8mm Bearing:5
- Flush:21: AA045:2 ↔ Steel Rod 8mm x 80mm:1
- Mate:709: AA034:1 ↔ AA045:2
- Mate:710: Steel Rod 8mm x 80mm:1 ↔ AASG09
- Mate:711: AA045:2 ↔ AASG09
- Mate:712: 12V DC Motor 378-1:3 ↔ AASG09
- Mate:713: AA045:2 ↔ AASG09
- Mate:714: 12V DC Motor 378-1:3 ↔ 4mm mounting hub:8
- Mate:715: AA045:2 ↔ 4mm mounting hub:8
- Mate:716: 4mm mounting hub:8 ↔ AASG09
- Mate:717: AA045:2 ↔ Bourns ACE 128:6
- Mate:718: AA045:2 ↔ Bourns ACE 128:6
- Angle:12 (0 deg): AA045:2 ↔ Bourns ACE 128:6
- Mate:719: AA045:2 ↔ 22x8x8mm Bearing:6
- Mate:720: AA045:2 ↔ 8mm Hub:8
- Mate:721: Steel Rod 8mm x 80mm:1 ↔ 8mm Hub:8
- Mate:722: Bourns ACE 128:6 ↔ AASG10
- Mate:723: AA045:2 ↔ AASG10
- Mate:724: Steel Rod 8mm x 80mm:1 ↔ AASG10
- Mate:725: AA045:2 ↔ AASG10
- Mate:726: 8mm Hub:8 ↔ AASG10
- Mate:727: AA046:1 ↔ 8mm Hub:9
- Mate:728: AA046:1 ↔ 8mm Hub:9
- Mate:730: Steel Rod 8mm x 80mm:1 ↔ 8mm Hub:9
- Mate:731: AA046:1 ↔ AASG09
- Mate:733: Servo Mounting Hub:1 ↔ MG995:1
- Mate:734: Servo Mounting Hub:1 ↔ MG995:1
- Mate:735: AA046:1 ↔ AA047:1
- Mate:736: AA046:1 ↔ AA047:1
- Mate:737: AA046:1 ↔ AA047:1
- Mate:738: AA047:1 ↔ Servo Mounting Hub:1
- Mate:739: AA047:1 ↔ Servo Mounting Hub:1
- Mate:740: AA047:1 ↔ Servo Mounting Hub:1
- Mate:742: AA043:3 ↔ Bourns ACE 128:6
- Mate:743: AA043:3 ↔ Bourns ACE 128:6
- Angle:13 (0 deg): AA043:3 ↔ AASG10
- Mate:744: AA048:1 ↔ MG995:1
- Mate:745 (0.5 mm): AA048:1 ↔ MG995:1
- Mate:746 (0.5 mm): AA048:1 ↔ MG995:1
- Mate:747: AA048:1 ↔ Gripper B Assembly:1
- Mate:748: AA048:1 ↔ Gripper B Assembly:1
- Mate:749: AA048:1 ↔ Gripper B Assembly:1
- Angle:14 (0 deg): AA042:1 ↔ AASG08
- Mate:751: AA008c:1 ↔ AA008d:1
- Mate:752: AA046:1 ↔ ISO 4018 M5 x 10:2
- Mate:753: AA047:1 ↔ ISO 4018 M5 x 10:2
- Mate:754: AA047:1 ↔ ISO 4018 M5 x 10:1
- Mate:755: AA047:1 ↔ ISO 4018 M5 x 10:1
- Mate:756: AA046:1 ↔ 8mm Hub:9
- Mate:757: AA046:1 ↔ AASG09
- Mate:758: AA046:1 ↔ ISO 4018 M5 x 25:1
- Mate:759: AA046:1 ↔ ISO 4018 M5 x 25:2
- Mate:760: AA046:1 ↔ ISO 4018 M5 x 25:3
- Mate:761: AA046:1 ↔ ISO 4018 M5 x 25:1
- Mate:762: AA046:1 ↔ ISO 4018 M5 x 25:3
- Mate:763: AA046:1 ↔ ISO 4018 M5 x 25:2
- Mate:764: 8mm Hub:9 ↔ ISO 7045 H M3 x 12 - 4.8 - H:3
- Mate:765: 8mm Hub:9 ↔ ISO 7045 H M3 x 12 - 4.8 - H:1
- Mate:766: 8mm Hub:9 ↔ ISO 7045 H M3 x 12 - 4.8 - H:2
- Mate:767: 8mm Hub:9 ↔ ISO 7045 H M3 x 12 - 4.8 - H:1
- Mate:768: 8mm Hub:9 ↔ ISO 7045 H M3 x 12 - 4.8 - H:2
- Mate:769: 8mm Hub:9 ↔ ISO 7045 H M3 x 12 - 4.8 - H:3
- Mate:770: AASG09 ↔ ISO 7045 H M3 x 12 - 4.8 - H:4
- Mate:771: AASG09 ↔ ISO 7045 H M3 x 12 - 4.8 - H:5
- Mate:772: AASG09 ↔ ISO 7045 H M3 x 12 - 4.8 - H:7
- Mate:773: AASG09 ↔ ISO 7045 H M3 x 12 - 4.8 - H:6
- Mate:774: AASG09 ↔ ISO 7045 H M3 x 12 - 4.8 - H:5
- Mate:775: AASG09 ↔ ISO 7045 H M3 x 12 - 4.8 - H:4
- Mate:776: AASG09 ↔ ISO 7045 H M3 x 12 - 4.8 - H:7
- Mate:777: AASG09 ↔ ISO 7045 H M3 x 12 - 4.8 - H:6
- Mate:778: 12V DC Motor 378-1:3 ↔ ISO 7045 H M3 x 8 - 4.8 - H:5
- Mate:779: 12V DC Motor 378-1:3 ↔ ISO 7045 H M3 x 8 - 4.8 - H:6
- Mate:780: AA045:2 ↔ ISO 7045 H M3 x 8 - 4.8 - H:5
- Mate:781: AA045:2 ↔ ISO 7045 H M3 x 8 - 4.8 - H:6
- Mate:782: 4mm mounting hub:8 ↔ AASG09
- Mate:783: AA049:1 ↔ Steel Rod 8mm x 80mm:1
- Mate:784: AA045:2 ↔ AA049:1
- Mate:785: AA045:2 ↔ AA049:1
- Mate:786: AA049:1 ↔ ISO 4018 M5 x 10:5
- Mate:787: AA049:1 ↔ ISO 4018 M5 x 10:3
- Mate:788: AA049:1 ↔ ISO 4018 M5 x 10:4
- Mate:789: AA049:1 ↔ ISO 4018 M5 x 10:5
- Mate:790: AA049:1 ↔ ISO 4018 M5 x 10:3
- Mate:791: AA049:1 ↔ ISO 4018 M5 x 10:4
- Mate:792: Servo Mounting Hub:1 ↔ ISO 7045 H M3 x 8 - 4.8 - H:9
- Mate:793: Servo Mounting Hub:1 ↔ ISO 7045 H M3 x 8 - 4.8 - H:10
- Mate:794: Servo Mounting Hub:1 ↔ ISO 7045 H M3 x 8 - 4.8 - H:8
- Mate:795: Servo Mounting Hub:1 ↔ ISO 7045 H M3 x 8 - 4.8 - H:7
- Mate:796: Servo Mounting Hub:1 ↔ ISO 7045 H M3 x 8 - 4.8 - H:9
- Mate:797: Servo Mounting Hub:1 ↔ ISO 7045 H M3 x 8 - 4.8 - H:10
- Mate:798: Servo Mounting Hub:1 ↔ ISO 7045 H M3 x 8 - 4.8 - H:8
- Mate:799: Servo Mounting Hub:1 ↔ ISO 7045 H M3 x 8 - 4.8 - H:7
- Mate:800: AA047:1 ↔ ISO 7045 H M3 x 8 - 4.8 - H:11
- Mate:801: AA047:1 ↔ ISO 7045 H M3 x 8 - 4.8 - H:11
- Mate:802: AA006b:1 ↔ ISO 4018 M5 x 25:7
- Mate:803: AA006b:1 ↔ ISO 4018 M5 x 25:7
- Mate:804: AA006b:1 ↔ ISO 4018 M5 x 25:8
- Mate:805: AA006b:1 ↔ ISO 4018 M5 x 25:8
- Mate:806: AA005b:1 ↔ ISO 4018 M5 x 25:9
- Mate:807: AA005b:1 ↔ ISO 4018 M5 x 25:10
- Mate:808: AA005b:1 ↔ ISO 4018 M5 x 25:9
- Mate:809: AA005b:1 ↔ ISO 4018 M5 x 25:10
- Mate:810: AASG01 ↔ ISO 4018 M5 x 25:12
- Mate:811: AASG01 ↔ ISO 4018 M5 x 25:13
- Mate:812: AASG01 ↔ ISO 4018 M5 x 25:11
- Mate:813: AASG01 ↔ ISO 4018 M5 x 25:15
- Mate:814: AASG01 ↔ ISO 4018 M5 x 25:14
- Mate:815: AASG01 ↔ ISO 4018 M5 x 25:16
- Mate:816: AASG01 ↔ ISO 4018 M5 x 25:12
- Mate:817: AASG01 ↔ ISO 4018 M5 x 25:14
- Mate:818: AASG01 ↔ ISO 4018 M5 x 25:16
- Mate:819: AASG01 ↔ ISO 4018 M5 x 25:15
- Mate:820: AASG01 ↔ ISO 4018 M5 x 25:11
- Mate:821: AASG01 ↔ ISO 4018 M5 x 25:13
- Mate:822: AASG05 ↔ ISO 4018 M5 x 25:22
- Mate:823: AASG05 ↔ ISO 4018 M5 x 25:17
- Mate:824: AASG05 ↔ ISO 4018 M5 x 25:18
- Mate:825: AASG05 ↔ ISO 4018 M5 x 25:19
- Mate:826: AA004:1 ↔ ISO 4018 M5 x 25:21
- Mate:827: AASG05 ↔ ISO 4018 M5 x 25:20
- Mate:828: AASG05 ↔ ISO 4018 M5 x 25:20
- Mate:829: AASG05 ↔ ISO 4018 M5 x 25:18
- Mate:830: AASG05 ↔ ISO 4018 M5 x 25:22
- Mate:831: AASG05 ↔ ISO 4018 M5 x 25:17
- Mate:832: AASG05 ↔ ISO 4018 M5 x 25:19
- Mate:833: AASG05 ↔ ISO 4018 M5 x 25:21
- Mate:834: AA001c:1 ↔ ISO 4018 M5 x 25:24
- Mate:835: AA001c:1 ↔ ISO 4018 M5 x 25:24
- Mate:836: AA001c:1 ↔ ISO 4018 M5 x 25:23
- Mate:837: AA001c:1 ↔ ISO 4018 M5 x 25:23
- Mate:838: AA005b:1 ↔ AA006b:1
- Mate:839: AASG02 ↔ ISO 4018 M5 x 25:25
- Mate:841: AASG02 ↔ ISO 4018 M5 x 25:27
- Mate:842: AASG02 ↔ ISO 4018 M5 x 25:28
- Mate:843: AASG02 ↔ ISO 4018 M5 x 25:28
- Mate:844: AASG02 ↔ ISO 4018 M5 x 25:27
- Mate:845: AASG02 ↔ ISO 4018 M5 x 25:25
- Mate:846: AA008d:1 ↔ ISO 4018 M5 x 40:1
- Mate:847: AA008d:1 ↔ ISO 4018 M5 x 40:2
- Mate:848: AA008d:1 ↔ ISO 4018 M5 x 40:1
- Mate:849: AA008d:1 ↔ ISO 4018 M5 x 40:2
- Mate:850: ISO 4035 M5:1 ↔ ISO 4018 M5 x 40:1
- Mate:851: AA035:1 ↔ ISO 4035 M5:1
- Mate:852: ISO 4035 M5:2 ↔ ISO 4018 M5 x 40:2
- Mate:853: AA035:1 ↔ ISO 4035 M5:2
- Mate:854: AA008d:1 ↔ ISO 4018 M5 x 25:29
- Mate:855: AA008d:1 ↔ ISO 4018 M5 x 25:32
- Mate:856: AA008d:1 ↔ ISO 4018 M5 x 25:30
- Mate:857: AA008d:1 ↔ ISO 4018 M5 x 25:31
- Flush:22 (12 mm): AA008d:1 ↔ ISO 4018 M5 x 25:31
- Flush:23 (-12 mm): AA008d:1 ↔ ISO 4018 M5 x 25:30
- Mate:858: AA008d:1 ↔ ISO 4018 M5 x 25:29
- Mate:859: AA008d:1 ↔ ISO 4018 M5 x 25:32
- Mate:860: AASG03 ↔ ISO 4018 M5 x 25:33
- Mate:861: AASG03 ↔ ISO 4018 M5 x 25:35
- Mate:862: AASG03 ↔ ISO 4018 M5 x 25:34
- Mate:863: AASG03 ↔ ISO 4018 M5 x 25:34
- Mate:864: AASG03 ↔ ISO 4018 M5 x 25:35
- Mate:865: AASG03 ↔ ISO 4018 M5 x 25:33
- Mate:866: AA037:1 ↔ ISO 4018 M5 x 35:1
- Mate:867: AA037:1 ↔ ISO 4018 M5 x 35:1
- Mate:868: AA036:1 ↔ ISO 4018 M5 x 35:2
- Flush:24: ISO 4018 M5 x 35:1 ↔ ISO 4018 M5 x 35:2
- Mate:869: ISO 4035 M5:3 ↔ ISO 4018 M5 x 35:1
- Mate:870: ISO 4035 M5:4 ↔ ISO 4018 M5 x 35:2
- Mate:871: AA036:1 ↔ ISO 4035 M5:4
- Mate:872: AA036:1 ↔ ISO 4035 M5:3
- Mate:873: AA037:1 ↔ ISO 4018 M5 x 25:39
- Mate:874: AA037:1 ↔ ISO 4018 M5 x 25:38
- Mate:875: AA037:1 ↔ ISO 4018 M5 x 25:37
- Mate:876: AA037:1 ↔ ISO 4018 M5 x 25:36
- Flush:25 (-9 mm): AA037:1 ↔ ISO 4018 M5 x 25:39
- Flush:26 (9 mm): AA037:1 ↔ ISO 4018 M5 x 25:38
- Mate:877: AA016b:1 ↔ ISO 4018 M5 x 25:37
- Mate:878: AA016b:1 ↔ ISO 4018 M5 x 25:36
- Mate:879: AA034:1 ↔ ISO 4018 M5 x 25:42
- Mate:880: AA034:1 ↔ ISO 4018 M5 x 25:41
- Mate:881: AA034:1 ↔ ISO 4018 M5 x 25:43
- Mate:882: AA034:1 ↔ ISO 4018 M5 x 25:40
- Mate:883: AA034:1 ↔ ISO 4018 M5 x 25:40
- Mate:884: AA034:1 ↔ ISO 4018 M5 x 25:43
- Mate:885: AA034:1 ↔ ISO 4018 M5 x 25:42
- Mate:886: AA034:1 ↔ ISO 4018 M5 x 25:41
- Mate:887: 4mm mounting hub:1 ↔ AASG01
- Mate:888: AASG01 ↔ ISO 7045 H M3 x 12 - 4.8 - H:9
- Mate:889: AASG01 ↔ ISO 7045 H M3 x 12 - 4.8 - H:8
- Mate:890: AASG01 ↔ ISO 7045 H M3 x 12 - 4.8 - H:8
- Mate:891: AASG01 ↔ ISO 7045 H M3 x 12 - 4.8 - H:9
- Mate:892: AA044:2 ↔ ISO 7045 H M3 x 8 - 4.8 - H:12
- Mate:893: AA044:2 ↔ ISO 7045 H M3 x 8 - 4.8 - H:12
- Mate:894: uxcell 12V 5RPM 8mm Worm Gear Motor:1 ↔ 8mm Hub:10
- Mate:895: AA001c:1 ↔ 8mm Hub:10
- Mate:896: 8mm Hub:10 ↔ AASG02
- Mate:897: AASG02 ↔ ISO 7045 H M3 x 8 - 4.8 - H:13
- Mate:898: AASG02 ↔ ISO 7045 H M3 x 8 - 4.8 - H:14
- Mate:899: AASG02 ↔ ISO 7045 H M3 x 8 - 4.8 - H:15
- Mate:900: AASG02 ↔ ISO 7045 H M3 x 8 - 4.8 - H:13
- Mate:901: AASG02 ↔ ISO 7045 H M3 x 8 - 4.8 - H:14
- Mate:902: AASG02 ↔ ISO 7045 H M3 x 8 - 4.8 - H:15
- Mate:903: uxcell 12V 5RPM 8mm Worm Gear Motor:1 ↔ ISO 4762 M4 x 10:1
- Mate:904: uxcell 12V 5RPM 8mm Worm Gear Motor:1 ↔ ISO 4762 M4 x 10:2
- Mate:905: AA001c:1 ↔ ISO 4762 M4 x 10:1
- Mate:906: AA001c:1 ↔ ISO 4762 M4 x 10:2
- Mate:907: 12V DC Motor 378-1:6 ↔ ISO 7045 H M3 x 8 - 4.8 - H:17
- Mate:908: 12V DC Motor 378-1:6 ↔ ISO 7045 H M3 x 8 - 4.8 - H:16
- Mate:909: AA005b:1 ↔ ISO 7045 H M3 x 8 - 4.8 - H:17
- Mate:910: AA005b:1 ↔ ISO 7045 H M3 x 8 - 4.8 - H:16
- Mate:911: 8mm Hub:6 ↔ ISO 7045 H M3 x 12 - 4.8 - H:10
- Mate:912: 8mm Hub:6 ↔ ISO 7045 H M3 x 12 - 4.8 - H:12
- Mate:913: 8mm Hub:6 ↔ ISO 7045 H M3 x 12 - 4.8 - H:11
- Mate:914: 8mm Hub:6 ↔ ISO 7045 H M3 x 12 - 4.8 - H:10
- Mate:915: 8mm Hub:6 ↔ ISO 7045 H M3 x 12 - 4.8 - H:11
- Mate:916: 8mm Hub:6 ↔ ISO 7045 H M3 x 12 - 4.8 - H:12
- Mate:917: AASG04 ↔ ISO 7045 H M3 x 12 - 4.8 - H:14
- Mate:918: AASG04 ↔ ISO 7045 H M3 x 12 - 4.8 - H:15
- Mate:919: AASG04 ↔ ISO 7045 H M3 x 12 - 4.8 - H:13
- Mate:920: AASG04 ↔ ISO 7045 H M3 x 12 - 4.8 - H:13
- Mate:921: AASG04 ↔ ISO 7045 H M3 x 12 - 4.8 - H:14
- Mate:922: AASG04 ↔ ISO 7045 H M3 x 12 - 4.8 - H:15
- Mate:923: 12V DC Motor 378-1:7 ↔ ISO 7045 H M3 x 8 - 4.8 - H:18
- Mate:924: 12V DC Motor 378-1:7 ↔ ISO 7045 H M3 x 8 - 4.8 - H:19
- Mate:925: AA008d:1 ↔ ISO 7045 H M3 x 8 - 4.8 - H:18
- Mate:926: AA008d:1 ↔ ISO 7045 H M3 x 8 - 4.8 - H:19
- Mate:927: AA010b:1 ↔ ISO 7045 H M3 x 12 - 4.8 - H:21
- Mate:928: AA010b:1 ↔ ISO 7045 H M3 x 12 - 4.8 - H:20
- Mate:929: AA010b:1 ↔ ISO 7045 H M3 x 12 - 4.8 - H:16
- Mate:930: AA010b:1 ↔ ISO 7045 H M3 x 12 - 4.8 - H:19
- Mate:931: AA010b:1 ↔ ISO 7045 H M3 x 12 - 4.8 - H:18
- Mate:932: AA010b:1 ↔ ISO 7045 H M3 x 12 - 4.8 - H:17
- Mate:933: 8mm Hub:3 ↔ ISO 7045 H M3 x 12 - 4.8 - H:19
- Mate:934: 8mm Hub:3 ↔ ISO 7045 H M3 x 12 - 4.8 - H:17
- Mate:935: 8mm Hub:3 ↔ ISO 7045 H M3 x 12 - 4.8 - H:18
- Mate:936: 8mm Hub:3 ↔ ISO 7045 H M3 x 12 - 4.8 - H:16
- Mate:937: 8mm Hub:3 ↔ ISO 7045 H M3 x 12 - 4.8 - H:20
- Mate:938: 8mm Hub:3 ↔ ISO 7045 H M3 x 12 - 4.8 - H:21
- Mate:939: AA036:1 ↔ ISO 4018 M5 x 25:33
- Mate:940: AASG03 ↔ ISO 7045 H M3 x 12 - 4.8 - H:24
- Mate:941: AASG03 ↔ ISO 7045 H M3 x 12 - 4.8 - H:23
- Mate:942: AASG03 ↔ ISO 7045 H M3 x 12 - 4.8 - H:22
- Mate:943: AASG03 ↔ ISO 7045 H M3 x 12 - 4.8 - H:22
- Mate:944: AASG03 ↔ ISO 7045 H M3 x 12 - 4.8 - H:23
- Mate:945: AASG03 ↔ ISO 7045 H M3 x 12 - 4.8 - H:24
- Mate:946: uxcell 12V 6RPM 6mm Worm Gear Motor:1 ↔ ISO 4762 M4 x 10:3
- Mate:947: uxcell 12V 6RPM 6mm Worm Gear Motor:1 ↔ ISO 4762 M4 x 10:4
- Mate:948: AA010b:1 ↔ ISO 4762 M4 x 10:4
- Mate:949: AA010b:1 ↔ ISO 4762 M4 x 10:3
- Mate:950: AA037:1 ↔ ISO 7045 H M3 x 8 - 4.8 - H:21
- Mate:951: AA037:1 ↔ ISO 7045 H M3 x 8 - 4.8 - H:20
- Mate:952: AA037:1 ↔ ISO 7045 H M3 x 8 - 4.8 - H:21
- Mate:953: AA037:1 ↔ ISO 7045 H M3 x 8 - 4.8 - H:20
- Mate:954: AA031:1 ↔ ISO 7045 H M3 x 8 - 4.8 - H:22
- Mate:955: AA031:1 ↔ ISO 7045 H M3 x 8 - 4.8 - H:23
- Mate:956: AA031:1 ↔ ISO 7045 H M3 x 8 - 4.8 - H:22
- Mate:957: AA031:1 ↔ ISO 7045 H M3 x 8 - 4.8 - H:23
- Mate:958: AASG07 ↔ ISO 7045 H M3 x 8 - 4.8 - H:25
- Mate:959: AASG07 ↔ ISO 7045 H M3 x 8 - 4.8 - H:26
- Mate:960: AASG07 ↔ ISO 7045 H M3 x 8 - 4.8 - H:24
- Mate:961: AASG07 ↔ ISO 7045 H M3 x 8 - 4.8 - H:26
- Mate:962: AASG07 ↔ ISO 7045 H M3 x 8 - 4.8 - H:25
- Mate:963: AASG07 ↔ ISO 7045 H M3 x 8 - 4.8 - H:24
- Mate:964: AA034:1 ↔ ISO 7045 H M3 x 8 - 4.8 - H:28
- Mate:965: AA034:1 ↔ ISO 7045 H M3 x 8 - 4.8 - H:27
- Mate:966: AA034:1 ↔ ISO 7045 H M3 x 8 - 4.8 - H:29
- Mate:967: AA034:1 ↔ ISO 7045 H M3 x 8 - 4.8 - H:30
- Mate:968: AA034:1 ↔ ISO 7045 H M3 x 8 - 4.8 - H:32
- Mate:969: AA034:1 ↔ ISO 7045 H M3 x 8 - 4.8 - H:31
- Mate:970: AA034:1 ↔ ISO 7045 H M3 x 8 - 4.8 - H:30
- Mate:971: AA034:1 ↔ ISO 7045 H M3 x 8 - 4.8 - H:29
- Mate:972: AA034:1 ↔ ISO 7045 H M3 x 8 - 4.8 - H:27
- Mate:973: AA034:1 ↔ ISO 7045 H M3 x 8 - 4.8 - H:28
- Mate:974: AA034:1 ↔ ISO 7045 H M3 x 8 - 4.8 - H:32
- Mate:975: AA034:1 ↔ ISO 7045 H M3 x 8 - 4.8 - H:31
- Mate:976: AA014:2 ↔ ISO 4017 M5 x 20:6
- Mate:977: AA014:2 ↔ ISO 4017 M5 x 20:5
- Mate:978: AA014:2 ↔ ISO 4017 M5 x 20:4
- Mate:979: AA014:2 ↔ ISO 4017 M5 x 20:5
- Mate:980: AA014:2 ↔ ISO 4017 M5 x 20:4
- Mate:981: AA014:2 ↔ ISO 4017 M5 x 20:6
